# Autodesk Inventor assembly: cellSTORM_v5_microsocpe
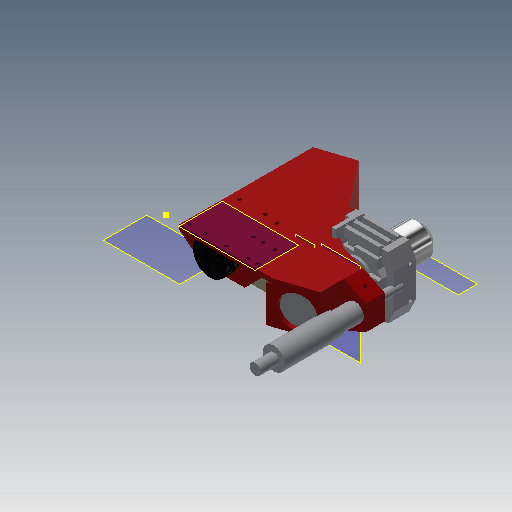
[picture p0: Inventor's stored thumbnail of the model, 512x512]
Saved by Autodesk Inventor 2019 (Build 230136000, 136)
## iProperties
Created: 2020-04-25
Part Number: cellSTORM_v5_microsocpe
Document SubType Name: Assembly
Designer: diederichbenedict
Author: diederichbenedict
## Documents named in this file (8)
- C:\Users\diederichbenedict\Dropbox\Dokumente\Promotion\PROJECTS\STORMoChip\GITHUB\CAD\Nanoscopy-on-the-cheap\Workspace\cellSTORM_v5_microsocpe.iam
- C:\Users\diederichbenedict\Dropbox\Dokumente\Promotion\PROJECTS\STORMoChip\GITHUB\CAD\Nanoscopy-on-the-cheap\Workspace\10_Filteslide_25mm.ipt
- C:\Users\diederichbenedict\Dropbox\Dokumente\Promotion\PROJECTS\STORMoChip\GITHUB\CAD\Nanoscopy-on-the-cheap\Workspace\00_Eyepiece_20x_WF.ipt
- C:\Users\diederichbenedict\Dropbox\Dokumente\Promotion\PROJECTS\STORMoChip\GITHUB\CAD\Nanoscopy-on-the-cheap\Workspace\cellSTORM_lightpath.ipt
- C:\Users\diederichbenedict\Dropbox\Dokumente\Promotion\PROJECTS\STORMoChip\GITHUB\CAD\Nanoscopy-on-the-cheap\Workspace\PF10-03-P01-Step.ipt
- C:\Users\diederichbenedict\Dropbox\Dokumente\Promotion\PROJECTS\STORMoChip\GITHUB\CAD\Nanoscopy-on-the-cheap\Workspace\cellSTORM_v5_opticalstage.ipt
- C:\Users\diederichbenedict\Dropbox\Dokumente\Promotion\PROJECTS\STORMoChip\GITHUB\CAD\Nanoscopy-on-the-cheap\Workspace\00_Micrometer.ipt
- C:\Users\diederichbenedict\Dropbox\Dokumente\Promotion\PROJECTS\STORMoChip\GITHUB\CAD\Nanoscopy-on-the-cheap\Workspace\Assembly_Z_stage.iam
## Components (8 placed, 7 different names)
1. 10_Filteslide_25mm:1
2. 00_Eyepiece_20x_WF:1
3. PF10-03-P01-Step:1
4. PF10-03-P01-Step:2
5. Assembly_Z_stage:1 [sub-assembly] — Insert:7
6. cellSTORM_v5_opticalstage:1 — Insert:6, Insert:7
7. cellSTORM_lightpath:1
8. 00_Micrometer:1 — Insert:6
## Relationships (6: Insert 6)
- [Insert]: PF10-03-P01-Step:1 ↔ cellSTORM_lightpath:1
- [Insert]: PF10-03-P01-Step:2 ↔ cellSTORM_lightpath:1
- [Insert] (40 mm): 10_Filteslide_25mm:1 ↔ cellSTORM_lightpath:1
- [Insert] (-10 mm): 00_Eyepiece_20x_WF:1 ↔ cellSTORM_lightpath:1
- Insert:6: cellSTORM_v5_opticalstage:1 ↔ 00_Micrometer:1
- Insert:7: Assembly_Z_stage:1 ↔ cellSTORM_v5_opticalstage:1
